# Autodesk Inventor assembly: SmallCardBox
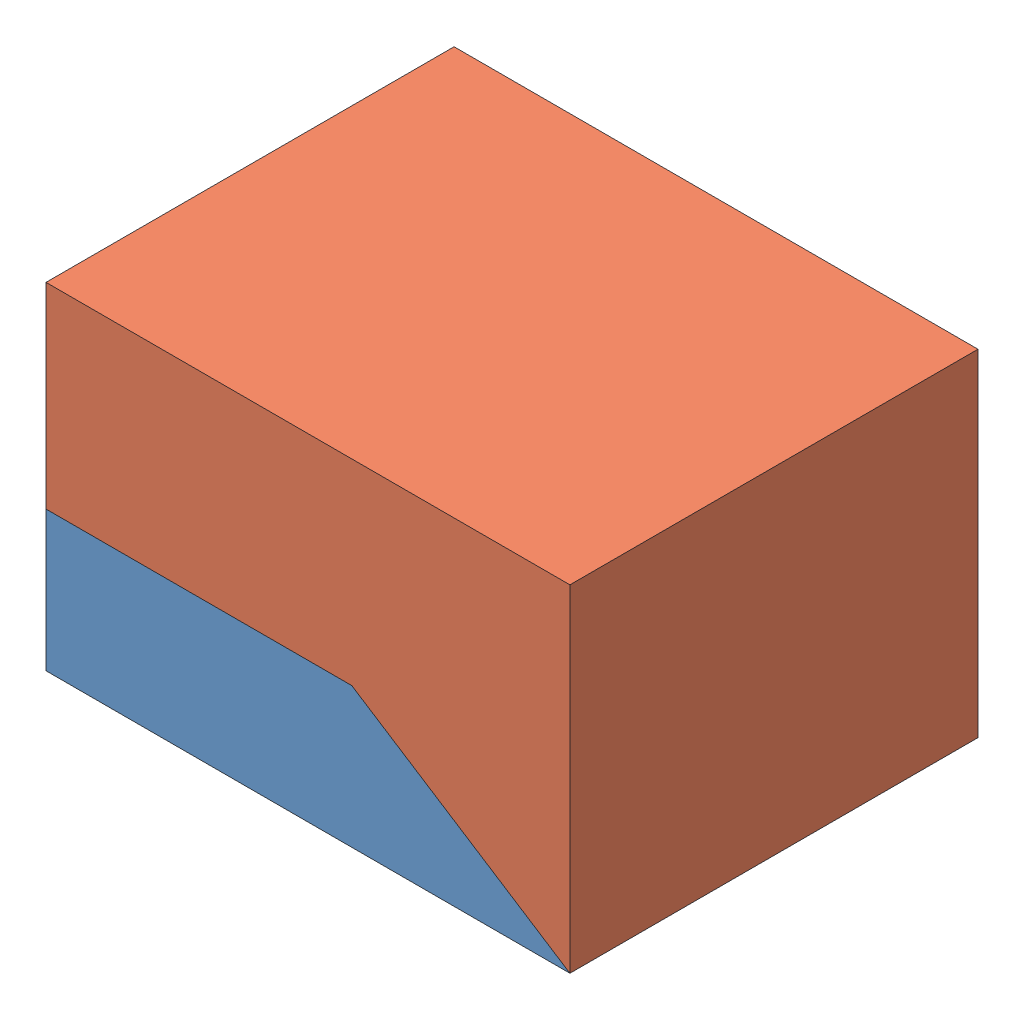
[picture p0: shaded view drawn from the shape stored in the file]
Saved by Autodesk Inventor 2022.2 (Build 262287010, 287A)
## iProperties
Created: 2022-07-12
Part Number: SmallCardBox
Document SubType Name: Assembly
Designer: keaton
Author: keaton
## Documents named in this file (1)
- C:\Users\keaton\Documents\3D Printing\KamigamiBox\SmallCardBox.iam
## Named parameters: test = 25.4 mm
